# Autodesk Inventor assembly: SQUICK_full
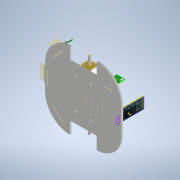
[picture p0: Inventor's stored thumbnail of the model, 180x180]
Saved by Autodesk Inventor 2020.3 (Build 243373000, 373)
## iProperties
Created: 2021-03-17
Part Number: SQUICK_full
Document SubType Name: Assembly
Designer: patry
Author: patry
## Documents named in this file (11)
- C:\Users\patry\Desktop\MM Squick\squick_inventor\Workspace\SQUICK_full.iam
- C:\Users\patry\Desktop\MM Squick\squick_inventor\Workspace\Board_base\board_base.ipt
- C:\Users\patry\Desktop\MM Squick\squick_inventor\Workspace\Motor with brace\micro-metal-gearmotor-extended-with-1089-extended-bracket.ipt
- C:\Users\patry\Desktop\MM Squick\squick_inventor\Workspace\Encoders\magnetic-encoder-pair-kit-for-micro-metal-gearmotors-hpcb-compatible\magnetic-encoder-pair-kit-for-micro-metal-gearmotors-hpcb-compatible-enc0.ipt
- C:\Users\patry\Desktop\MM Squick\squick_inventor\Workspace\Encoders\magnetic-encoder-pair-kit-for-micro-metal-gearmotors-hpcb-compatible\magnetic-encoder-pair-kit-for-micro-metal-gearmotors-hpcb-compatible-w1r0.ipt
- C:\Users\patry\Desktop\MM Squick\squick_inventor\Workspace\PINS\GCT_BF02106AB04000280NG\AIS2020\BF021-06-A-B-0400-0280-N-G.iam
- C:\Users\patry\Desktop\MM Squick\squick_inventor\Workspace\BT_Module\BLUTOOTH.ipt
- C:\Users\patry\Desktop\MM Squick\squick_inventor\Workspace\Power\pololu-2843-step-down-regulator-5-volt-1.snapshot.2\Pololu 2843 5V Step Down Regulator.ipt
- C:\Users\patry\Desktop\MM Squick\squick_inventor\Workspace\PINS\single-row-male-pin-headers-1.snapshot.3\1x4 Male Pin Header Angle.ipt
- C:\Users\patry\Desktop\MM Squick\squick_inventor\Workspace\VL\vl53l0x-vl53l1x-vl53l3cx-carrier-model.ipt
- C:\Users\patry\Desktop\MM Squick\squick_inventor\Workspace\PINS\single-row-male-pin-headers-1.snapshot.3\1x7 Male Pin Header Angle.ipt
## Components (18 placed, 10 different names)
1. board_base:1 — Zestawiające:1, Zestawiające:2, Równoległe:1, Równoległe:2, Zestawiające:3, Zestawiające:4, Kątowe:1, Kątowe:2, Zestawiające:16, Kątowe:5, Zestawiające:18, Kątowe:6, Zestawiające:20, Zestawiające:21, Zestawiające:24, Kątowe:7, Kątowe:8, Zestawiające:26, Zestawiające:28, Kątowe:9
2. micro-metal-gearmotor-extended-with-1089-extended-bracket:1 — Zestawiające:1, Równoległe:1, Zestawiające:4, Zestawiające:5, Zestawiające:7, Zestawiające:8
3. micro-metal-gearmotor-extended-with-1089-extended-bracket:2 — Zestawiające:2, Równoległe:2, Zestawiające:3, Zestawiające:6, Zestawiające:10, Zestawiające:13
4. magnetic-encoder-pair-kit-for-micro-metal-gearmotors-hpcb-compatible-enc0:1 — Zestawiające:7, Zestawiające:8, Zestawiające:9, Kątowe:1, Zestawiające:12, Zestawiające:19
5. magnetic-encoder-pair-kit-for-micro-metal-gearmotors-hpcb-compatible-w1r0:1 — Zestawiające:5, Zestawiające:9, Zestawiające:12
6. magnetic-encoder-pair-kit-for-micro-metal-gearmotors-hpcb-compatible-enc0:2 — Zestawiające:10, Kątowe:2, Zestawiające:11, Zestawiające:13, Zestawiające:22
7. magnetic-encoder-pair-kit-for-micro-metal-gearmotors-hpcb-compatible-w1r0:2 — Zestawiające:6, Zestawiające:11
8. BF021-06-A-B-0400-0280-N-G:1 [sub-assembly] — Zestawiające:19, Zestawiające:20
9. BLUTOOTH:1 — Zestawiające:16, Kątowe:5
10. Pololu 2843 5V Step Down Regulator:1 — Zestawiające:17, Równoległe:3, Równoległe:4, Zestawiające:18, Kątowe:6
11. 1x4 Male Pin Header Angle:1 — Zestawiające:17, Równoległe:3, Równoległe:4
12. BF021-06-A-B-0400-0280-N-G:2 [sub-assembly] — Zestawiające:21, Zestawiające:22
13. vl53l0x-vl53l1x-vl53l3cx-carrier-model:1 — Zestawiające:23, Równoległe:5, Równoległe:6, Kątowe:7
14. 1x7 Male Pin Header Angle:2 — Zestawiające:23, Równoległe:5, Równoległe:6, Zestawiające:24
15. vl53l0x-vl53l1x-vl53l3cx-carrier-model:2 — Kątowe:8
16. 1x7 Male Pin Header Angle:3 — Zestawiające:26
17. vl53l0x-vl53l1x-vl53l3cx-carrier-model:3 — Kątowe:9
18. 1x7 Male Pin Header Angle:4 — Zestawiające:28
## Relationships (43: Mate 26, Flush 10, Angle 7)
- Zestawiające:1 [Mate] (0.75 mm): board_base:1 ↔ micro-metal-gearmotor-extended-with-1089-extended-bracket:1
- Zestawiające:2 [Mate] (0.75 mm): board_base:1 ↔ micro-metal-gearmotor-extended-with-1089-extended-bracket:2
- Równoległe:1 [Flush] (-0.5 mm): board_base:1 ↔ micro-metal-gearmotor-extended-with-1089-extended-bracket:1
- Równoległe:2 [Flush] (-0.5 mm): board_base:1 ↔ micro-metal-gearmotor-extended-with-1089-extended-bracket:2
- Zestawiające:3 [Mate]: board_base:1 ↔ micro-metal-gearmotor-extended-with-1089-extended-bracket:2
- Zestawiające:4 [Mate]: board_base:1 ↔ micro-metal-gearmotor-extended-with-1089-extended-bracket:1
- Zestawiające:5 [Mate]: micro-metal-gearmotor-extended-with-1089-extended-bracket:1 ↔ magnetic-encoder-pair-kit-for-micro-metal-gearmotors-hpcb-compatible-w1r0:1
- Zestawiające:6 [Mate]: micro-metal-gearmotor-extended-with-1089-extended-bracket:2 ↔ magnetic-encoder-pair-kit-for-micro-metal-gearmotors-hpcb-compatible-w1r0:2
- Zestawiające:7 [Mate]: micro-metal-gearmotor-extended-with-1089-extended-bracket:1 ↔ magnetic-encoder-pair-kit-for-micro-metal-gearmotors-hpcb-compatible-enc0:1
- Zestawiające:8 [Mate]: micro-metal-gearmotor-extended-with-1089-extended-bracket:1 ↔ magnetic-encoder-pair-kit-for-micro-metal-gearmotors-hpcb-compatible-enc0:1
- Zestawiające:9 [Mate] (0.5 mm): magnetic-encoder-pair-kit-for-micro-metal-gearmotors-hpcb-compatible-enc0:1 ↔ magnetic-encoder-pair-kit-for-micro-metal-gearmotors-hpcb-compatible-w1r0:1
- Kątowe:1 [Angle] (180 deg): board_base:1 ↔ magnetic-encoder-pair-kit-for-micro-metal-gearmotors-hpcb-compatible-enc0:1
- Zestawiające:10 [Mate]: micro-metal-gearmotor-extended-with-1089-extended-bracket:2 ↔ magnetic-encoder-pair-kit-for-micro-metal-gearmotors-hpcb-compatible-enc0:2
- Kątowe:2 [Angle] (180 deg): board_base:1 ↔ magnetic-encoder-pair-kit-for-micro-metal-gearmotors-hpcb-compatible-enc0:2
- Zestawiające:11 [Mate] (0.5 mm): magnetic-encoder-pair-kit-for-micro-metal-gearmotors-hpcb-compatible-enc0:2 ↔ magnetic-encoder-pair-kit-for-micro-metal-gearmotors-hpcb-compatible-w1r0:2
- Zestawiające:12 [Mate] (0.5 mm): magnetic-encoder-pair-kit-for-micro-metal-gearmotors-hpcb-compatible-enc0:1 ↔ magnetic-encoder-pair-kit-for-micro-metal-gearmotors-hpcb-compatible-w1r0:1
- Zestawiające:13 [Mate]: micro-metal-gearmotor-extended-with-1089-extended-bracket:2 ↔ magnetic-encoder-pair-kit-for-micro-metal-gearmotors-hpcb-compatible-enc0:2
- Zestawiające:16 [Mate]: board_base:1 ↔ BLUTOOTH:1
- Kątowe:5 [Angle] (180 deg): board_base:1 ↔ BLUTOOTH:1
- Zestawiające:17 [Mate]: Pololu 2843 5V Step Down Regulator:1 ↔ 1x4 Male Pin Header Angle:1
- Równoległe:3 [Flush]: Pololu 2843 5V Step Down Regulator:1 ↔ 1x4 Male Pin Header Angle:1
- Równoległe:4 [Flush] (0.15 mm): Pololu 2843 5V Step Down Regulator:1 ↔ 1x4 Male Pin Header Angle:1
- Zestawiające:18 [Mate]: board_base:1 ↔ Pololu 2843 5V Step Down Regulator:1
- Kątowe:6 [Angle] (0 deg): board_base:1 ↔ Pololu 2843 5V Step Down Regulator:1
- Zestawiające:19 [Mate]: magnetic-encoder-pair-kit-for-micro-metal-gearmotors-hpcb-compatible-enc0:1 ↔ BF021-06-A-B-0400-0280-N-G:1
- Zestawiające:20 [Mate]: board_base:1 ↔ BF021-06-A-B-0400-0280-N-G:1
- Zestawiające:21 [Mate]: board_base:1 ↔ BF021-06-A-B-0400-0280-N-G:2
- Zestawiające:22 [Mate]: magnetic-encoder-pair-kit-for-micro-metal-gearmotors-hpcb-compatible-enc0:2 ↔ BF021-06-A-B-0400-0280-N-G:2
- Zestawiające:23 [Mate]: vl53l0x-vl53l1x-vl53l3cx-carrier-model:1 ↔ 1x7 Male Pin Header Angle:2
- Równoległe:5 [Flush]: vl53l0x-vl53l1x-vl53l3cx-carrier-model:1 ↔ 1x7 Male Pin Header Angle:2
- Równoległe:6 [Flush]: vl53l0x-vl53l1x-vl53l3cx-carrier-model:1 ↔ 1x7 Male Pin Header Angle:2
- Zestawiające:24 [Mate]: board_base:1 ↔ 1x7 Male Pin Header Angle:2
- Kątowe:7 [Angle] (0 deg): board_base:1 ↔ vl53l0x-vl53l1x-vl53l3cx-carrier-model:1
- [Mate]: vl53l0x-vl53l1x-vl53l3cx-carrier-model:2 ↔ 1x7 Male Pin Header Angle:3
- [Flush]: vl53l0x-vl53l1x-vl53l3cx-carrier-model:2 ↔ 1x7 Male Pin Header Angle:3
- [Flush]: vl53l0x-vl53l1x-vl53l3cx-carrier-model:2 ↔ 1x7 Male Pin Header Angle:3
- Kątowe:8 [Angle] (45 deg): board_base:1 ↔ vl53l0x-vl53l1x-vl53l3cx-carrier-model:2
- Zestawiające:26 [Mate]: board_base:1 ↔ 1x7 Male Pin Header Angle:3
- [Mate]: vl53l0x-vl53l1x-vl53l3cx-carrier-model:3 ↔ 1x7 Male Pin Header Angle:4
- [Flush]: vl53l0x-vl53l1x-vl53l3cx-carrier-model:3 ↔ 1x7 Male Pin Header Angle:4
- [Flush]: vl53l0x-vl53l1x-vl53l3cx-carrier-model:3 ↔ 1x7 Male Pin Header Angle:4
- Zestawiające:28 [Mate]: board_base:1 ↔ 1x7 Male Pin Header Angle:4
- Kątowe:9 [Angle] (-45 deg): board_base:1 ↔ vl53l0x-vl53l1x-vl53l3cx-carrier-model:3
## Named parameters: d44_d39 = 0 mm, d45_d40 = 0 mm, d46_d41 = 0 mm, d49_d39 = 0 mm, d50_d40 = 0 mm, d51_d41 = 0 mm
